# Autodesk Inventor assembly: mesa_suporte_de_placa
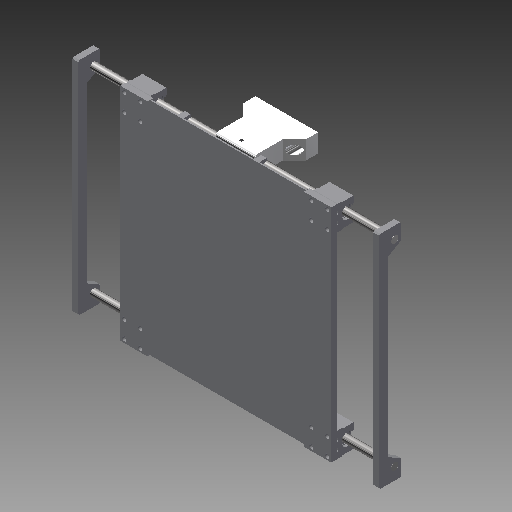
[picture p0: Inventor's stored thumbnail of the model, 512x512]
Saved by Autodesk Inventor 2018 (Build 220112000, 112)
## iProperties
Created: 2018-05-17
Part Number: mesa_suporte_de_placa
Material: Genérico
Document SubType Name: Assembly
Designer: Usuario
Mass: 2681.39 g
Surface Area: 5192.59 cm^2
Volume: 1283.96 cm^3
Density: 2.08838 g/cm^3
Author: Usuario
## Documents named in this file (8)
- C:\Users\Usuario\Desktop\pecas_3d-20180530T120808Z-001\pecas_3d\mesa_suporte_de_placa.iam
- C:\Users\Usuario\Desktop\pecas_3d-20180530T120808Z-001\pecas_3d\suporte_guia_central.ipt
- C:\Users\Usuario\Desktop\pecas_3d-20180530T120808Z-001\pecas_3d\guia_linear_12mm.ipt
- C:\Users\Usuario\Desktop\pecas_3d-20180530T120808Z-001\pecas_3d\SBR12UU.iam
- C:\Users\Usuario\Desktop\pecas_3d-20180530T120808Z-001\pecas_3d\EsbarrosCarro.ipt
- C:\Users\Usuario\Desktop\pecas_3d-20180530T120808Z-001\pecas_3d\SuportePincas.ipt
- C:\Users\Usuario\Desktop\pecas_3d-20180530T120808Z-001\pecas_3d\SuporteAntiEmpenamento.ipt
- C:\Users\Usuario\Desktop\pecas_3d-20180530T120808Z-001\pecas_3d\Peça1.ipt
## Components (15 placed, 7 different names)
1. suporte_guia_central:1 — Coincidência:1, Alinhamento:1, Alinhamento:2, Coincidência:2, Alinhamento:4
2. suporte_guia_central:2 — Coincidência:1, Alinhamento:1, Alinhamento:2, Coincidência:3, Alinhamento:6
3. guia_linear_12mm:1 — Coincidência:2, Alinhamento:4, Coincidência:4, Coincidência:27, Coincidência:28, Coincidência:31, Coincidência:33, Coincidência:36, Coincidência:40, Alinhamento:28
4. guia_linear_12mm:2 — Coincidência:3, Alinhamento:6, Coincidência:4, Coincidência:29, Coincidência:30, Coincidência:32, Alinhamento:23, Coincidência:34, Coincidência:35, Coincidência:39
5. SBR12UU:1 [sub-assembly] — Coincidência:28, Alinhamento:18, Alinhamento:19, Coincidência:38, Alinhamento:26, Alinhamento:27
6. SBR12UU:2 [sub-assembly] — Coincidência:29, Alinhamento:18, Alinhamento:19
7. SBR12UU:3 [sub-assembly] — Coincidência:27, Alinhamento:20, Alinhamento:21, Coincidência:37, Alinhamento:24, Alinhamento:25
8. SBR12UU:4 [sub-assembly] — Coincidência:30, Alinhamento:20, Alinhamento:21
9. EsbarrosCarro:2 — Coincidência:31, Coincidência:32, Alinhamento:23
10. SuporteAntiEmpenamento:1 — Coincidência:33, Coincidência:34
11. SuporteAntiEmpenamento:2 — Coincidência:35, Coincidência:36
12. SuportePincas:2 — Coincidência:38, Alinhamento:26, Alinhamento:27
13. SuportePincas:3 — Coincidência:37, Alinhamento:24, Alinhamento:25, Alinhamento:29
14. EsbarrosCarro:3 — Coincidência:39, Coincidência:40, Alinhamento:28
15. PCB — Alinhamento:29
## Relationships (33: Mate 18, Flush 15)
- Coincidência:1 [Mate] (290 mm): suporte_guia_central:1 ↔ suporte_guia_central:2
- Alinhamento:1 [Flush]: suporte_guia_central:1 ↔ suporte_guia_central:2
- Alinhamento:2 [Flush]: suporte_guia_central:1 ↔ suporte_guia_central:2
- Coincidência:2 [Mate]: suporte_guia_central:1 ↔ guia_linear_12mm:1
- Alinhamento:4 [Flush] (-217.8645 mm): suporte_guia_central:1 ↔ guia_linear_12mm:1
- Coincidência:3 [Mate]: suporte_guia_central:2 ↔ guia_linear_12mm:2
- Alinhamento:6 [Flush] (-217.8645 mm): suporte_guia_central:2 ↔ guia_linear_12mm:2
- Coincidência:4 [Mate]: guia_linear_12mm:1 ↔ guia_linear_12mm:2
- Coincidência:27 [Mate]: guia_linear_12mm:1 ↔ SBR12UU:3
- Coincidência:28 [Mate]: guia_linear_12mm:1 ↔ SBR12UU:1
- Coincidência:29 [Mate]: guia_linear_12mm:2 ↔ SBR12UU:2
- Coincidência:30 [Mate]: guia_linear_12mm:2 ↔ SBR12UU:4
- Alinhamento:18 [Flush]: SBR12UU:1 ↔ SBR12UU:2
- Alinhamento:19 [Flush]: SBR12UU:1 ↔ SBR12UU:2
- Alinhamento:20 [Flush]: SBR12UU:3 ↔ SBR12UU:4
- Alinhamento:21 [Flush]: SBR12UU:3 ↔ SBR12UU:4
- Coincidência:31 [Mate]: guia_linear_12mm:1 ↔ EsbarrosCarro:2
- Coincidência:32 [Mate]: guia_linear_12mm:2 ↔ EsbarrosCarro:2
- Alinhamento:23 [Flush]: guia_linear_12mm:2 ↔ EsbarrosCarro:2
- Coincidência:33 [Mate]: guia_linear_12mm:1 ↔ SuporteAntiEmpenamento:1
- Coincidência:34 [Mate]: guia_linear_12mm:2 ↔ SuporteAntiEmpenamento:1
- Coincidência:35 [Mate]: guia_linear_12mm:2 ↔ SuporteAntiEmpenamento:2
- Coincidência:36 [Mate]: guia_linear_12mm:1 ↔ SuporteAntiEmpenamento:2
- Coincidência:37 [Mate]: SBR12UU:3 ↔ SuportePincas:3
- Alinhamento:24 [Flush]: SBR12UU:3 ↔ SuportePincas:3
- Alinhamento:25 [Flush]: SBR12UU:3 ↔ SuportePincas:3
- Coincidência:38 [Mate]: SBR12UU:1 ↔ SuportePincas:2
- Alinhamento:26 [Flush]: SBR12UU:1 ↔ SuportePincas:2
- Alinhamento:27 [Flush]: SBR12UU:1 ↔ SuportePincas:2
- Coincidência:39 [Mate]: guia_linear_12mm:2 ↔ EsbarrosCarro:3
- Coincidência:40 [Mate]: guia_linear_12mm:1 ↔ EsbarrosCarro:3
- Alinhamento:28 [Flush]: guia_linear_12mm:1 ↔ EsbarrosCarro:3
- Alinhamento:29 [Flush]: SuportePincas:3 ↔ PCB
